# Autodesk Inventor assembly: M3_kužel_alien.ipt
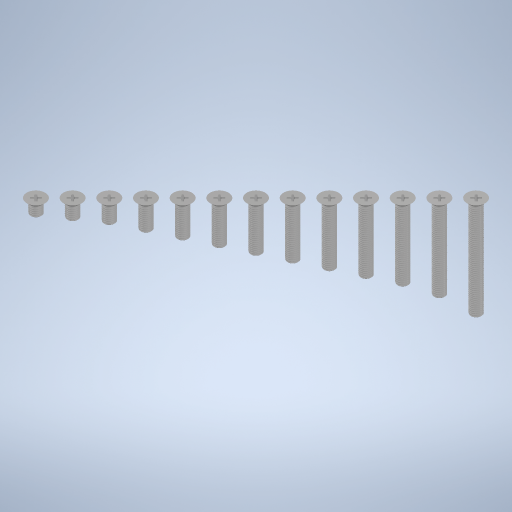
[picture p0: Inventor's stored thumbnail of the model, 512x512]
Saved by Autodesk Inventor 2023 (Build 270158000, 158)
## iProperties
Created: 2023-05-17
Part Number: M3_kužel_alien.ipt
Document SubType Name: Assembly
Designer: Simak
Author: Simak
## Documents named in this file (14)
- C:\Users\Simak\OneDrive\Plocha\3D modely\_Součástky\Šrouby\M3_kužel_philips\M3_kužel_alien.ipt.iam
- C:\Users\Simak\OneDrive\Plocha\3D modely\_Součástky\Šrouby\M3_kužel_philips\M3x4_kožel_alien.ipt
- C:\Users\Simak\OneDrive\Plocha\3D modely\_Součástky\Šrouby\M3_kužel_philips\M3x5_kožel_alien.ipt
- C:\Users\Simak\OneDrive\Plocha\3D modely\_Součástky\Šrouby\M3_kužel_philips\M3x6_kužel_alien.ipt
- C:\Users\Simak\OneDrive\Plocha\3D modely\_Součástky\Šrouby\M3_kužel_philips\M3x8_kužel_alien.ipt
- C:\Users\Simak\OneDrive\Plocha\3D modely\_Součástky\Šrouby\M3_kužel_philips\M3x10_kužel_alien.ipt
- C:\Users\Simak\OneDrive\Plocha\3D modely\_Součástky\Šrouby\M3_kužel_philips\M3x12_kužel_alien.ipt
- C:\Users\Simak\OneDrive\Plocha\3D modely\_Součástky\Šrouby\M3_kužel_philips\M3x14_kužel_alien.ipt
- C:\Users\Simak\OneDrive\Plocha\3D modely\_Součástky\Šrouby\M3_kužel_philips\M3x16_kužel_alien.ipt
- C:\Users\Simak\OneDrive\Plocha\3D modely\_Součástky\Šrouby\M3_kužel_philips\M3x18_kužel_alien.ipt
- C:\Users\Simak\OneDrive\Plocha\3D modely\_Součástky\Šrouby\M3_kužel_philips\M3x20_kužel_alien.ipt
- C:\Users\Simak\OneDrive\Plocha\3D modely\_Součástky\Šrouby\M3_kužel_philips\M3x22_kužel_alien.ipt
- C:\Users\Simak\OneDrive\Plocha\3D modely\_Součástky\Šrouby\M3_kužel_philips\M3x24_kužel_alien.ipt
- C:\Users\Simak\OneDrive\Plocha\3D modely\_Součástky\Šrouby\M3_kužel_philips\M3x26_kužel_alien.ipt
## Components (13 placed, 13 different names)
1. M3x4_kožel_alien:1 — Stejný směr:1, Stejný směr:2, Stejný směr:3, Stejný směr:4, Stejný směr:5, Stejný směr:6, Stejný směr:7, Stejný směr:8, Stejný směr:9, Stejný směr:10, Stejný směr:11, Stejný směr:12
2. M3x5_kožel_alien:1 — Stejný směr:1
3. M3x6_kužel_alien:1 — Stejný směr:2
4. M3x8_kužel_alien:1 — Stejný směr:3
5. M3x10_kužel_alien:1 — Stejný směr:4
6. M3x12_kužel_alien:1 — Stejný směr:5
7. M3x14_kužel_alien:1 — Stejný směr:6
8. M3x16_kužel_alien:1 — Stejný směr:7
9. M3x18_kužel_alien:1 — Stejný směr:8
10. M3x20_kužel_alien:1 — Stejný směr:9
11. M3x22_kužel_alien:1 — Stejný směr:10
12. M3x24_kužel_alien:1 — Stejný směr:11
13. M3x26_kužel_alien:1 — Stejný směr:12
## Relationships (12: Flush 12)
- Stejný směr:1 [Flush]: M3x4_kožel_alien:1 ↔ M3x5_kožel_alien:1
- Stejný směr:2 [Flush]: M3x4_kožel_alien:1 ↔ M3x6_kužel_alien:1
- Stejný směr:3 [Flush]: M3x4_kožel_alien:1 ↔ M3x8_kužel_alien:1
- Stejný směr:4 [Flush]: M3x4_kožel_alien:1 ↔ M3x10_kužel_alien:1
- Stejný směr:5 [Flush]: M3x4_kožel_alien:1 ↔ M3x12_kužel_alien:1
- Stejný směr:6 [Flush]: M3x4_kožel_alien:1 ↔ M3x14_kužel_alien:1
- Stejný směr:7 [Flush]: M3x4_kožel_alien:1 ↔ M3x16_kužel_alien:1
- Stejný směr:8 [Flush]: M3x4_kožel_alien:1 ↔ M3x18_kužel_alien:1
- Stejný směr:9 [Flush]: M3x4_kožel_alien:1 ↔ M3x20_kužel_alien:1
- Stejný směr:10 [Flush]: M3x4_kožel_alien:1 ↔ M3x22_kužel_alien:1
- Stejný směr:11 [Flush]: M3x4_kožel_alien:1 ↔ M3x24_kužel_alien:1
- Stejný směr:12 [Flush]: M3x4_kožel_alien:1 ↔ M3x26_kužel_alien:1
